# Autodesk Inventor assembly: шевронное очко
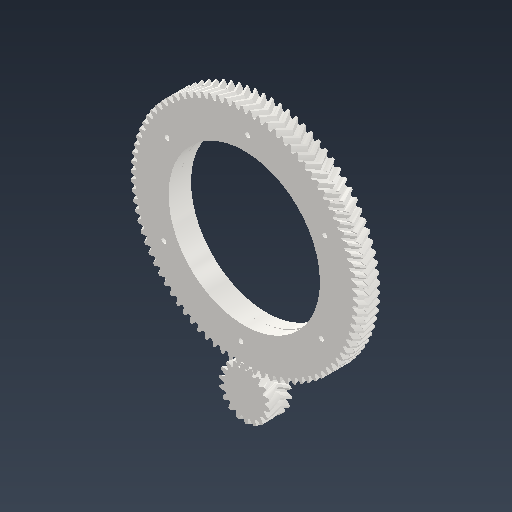
[picture p0: Inventor's stored thumbnail of the model, 512x512]
Saved by Autodesk Inventor 2026 (Build 300175000, 175)
## iProperties
Created: 2025-11-26
Part Number: шевронное очко
Document SubType Name: Assembly
Designer: Phantom
Author: Phantom
## Documents named in this file (3)
- C:\Users\GameHD\Desktop\Phantom 16950\шевронное очко.iam
- C:\Users\GameHD\Desktop\Phantom 16950\шевронное очко\Мастер проектирования\Цилиндрическое зубчатое зацепление1.iam
- C:\Users\GameHD\Desktop\Phantom 16950\шевронное очко\Мастер проектирования\Цилиндрическое зубчатое зацепление1_MIR.iam
## Components (2 placed, 2 different names)
1. Цилиндрическое зубчатое зацепление:1 [sub-assembly] — Совмещение:2, Совмещение:3, Совмещение:4
2. Цилиндрическое зубчатое зацепление1_MIR:1 [sub-assembly] — Совмещение:2, Совмещение:3, Совмещение:4
## Relationships (3: Mate 3)
- Совмещение:2 [Mate]: Цилиндрическое зубчатое зацепление:1 ↔ Цилиндрическое зубчатое зацепление1_MIR:1
- Совмещение:3 [Mate]: Цилиндрическое зубчатое зацепление:1 ↔ Цилиндрическое зубчатое зацепление1_MIR:1
- Совмещение:4 [Mate]: Цилиндрическое зубчатое зацепление:1 ↔ Цилиндрическое зубчатое зацепление1_MIR:1
